# Autodesk Inventor assembly: Ring
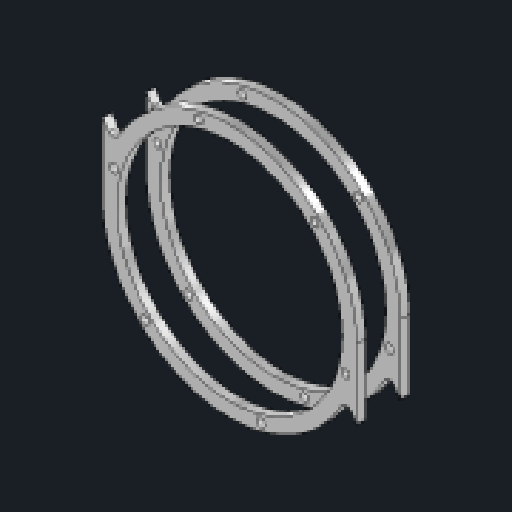
[picture p0: Inventor's stored thumbnail of the model, 512x512]
Saved by Autodesk Inventor 2023.2 (Build 272271030, 271C)
## iProperties
Created: 2024-03-01
Part Number: Ring
Document SubType Name: Assembly
Designer: robpl
Author: robpl
## Documents named in this file (3)
- C:\Users\robpl\OneDrive\Documents\Arduino\Onslaught\CAD\Onslaught V2\Ring.iam
- C:\Users\robpl\OneDrive\Documents\Arduino\Onslaught\CAD\Onslaught V2\Weapon.ipt
- C:\Users\robpl\OneDrive\Documents\Arduino\Onslaught\CAD\Onslaught V2\Pin.ipt
## Components (8 placed, 2 different names)
1. Weapon:1 — Mate:1, Mate:2, Mate:3
2. Weapon:2 — Mate:1, Mate:2, Mate:3, Mate:4, Flush:1
3. Pin:1 — Mate:4, Flush:1
4. Pin:2
5. Pin:3
6. Pin:4
7. Pin:5
8. Pin:6
## Component patterns: (6 elements, first: Pin:1)
## Relationships (5: Mate 4, Flush 1)
- Mate:1: Weapon:1 ↔ Weapon:2
- Mate:2: Weapon:1 ↔ Weapon:2
- Mate:3 (-29.6 mm): Weapon:1 ↔ Weapon:2
- Mate:4: Weapon:2 ↔ Pin:1
- Flush:1: Weapon:2 ↔ Pin:1
